# Autodesk Inventor assembly: final_Toolhead
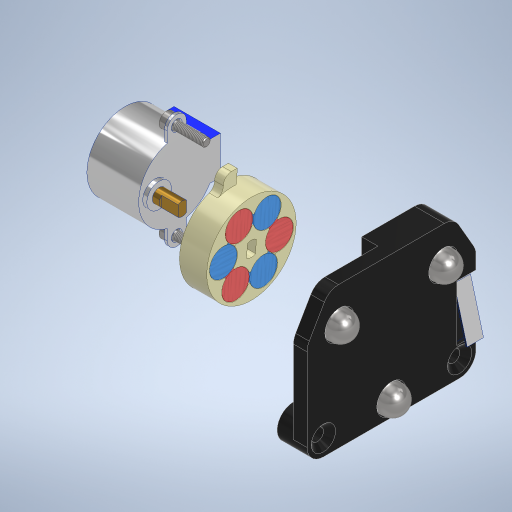
[picture p0: Inventor's stored thumbnail of the model, 512x512]
Saved by Autodesk Inventor 2023.2 (Build 272271000, 271)
## iProperties
Created: 2022-09-02
Part Number: final_Toolhead
Document SubType Name: Assembly
Designer: Remo
Author: Remo
## Documents named in this file (11)
- C:\Users\remop\OneDrive\Documents\Inventor\3D Printers\LuEVO\Mk4_Toolchanger\final_Toolhead.iam
- C:\Users\remop\OneDrive\Documents\Inventor\3D Printers\LuEVO\Mk4_Toolchanger\MagToolChanger_Lockplate.ipt
- C:\Users\remop\OneDrive\Documents\Inventor\3D Printers\LuEVO\Mk4_Toolchanger\MagToolChanger_HeadBase.ipt
- C:\Users\remop\OneDrive\Documents\Inventor\3D Printers\LuEVO\Mk4_Toolchanger\MagToolChanger_Motor.ipt
- C:\Users\remop\OneDrive\Documents\Inventor\3D Printers\LuEVO\Mk4_Toolchanger\MagToolChanger_RefSwitch.ipt
- C:\Users\remop\OneDrive\Documents\Inventor\3D Printers\LuEVO\Mk4_Toolchanger\MagToolChanger_Magnet.ipt
- C:\Users\remop\OneDrive\Documents\Inventor\3D Printers\LuEVO\Mk4_Toolchanger\MagToolChanger_CouplerBall.ipt
- C:\Users\remop\OneDrive\Documents\Inventor\Content Center Files\R2023\en-US\AS 1420\AS 1420 - 1973 - M3 x 12.ipt
- C:\Users\remop\OneDrive\Documents\Inventor\Content Center Files\R2023\en-US\ANSI B18.3.1M(6)\ANSI B18.3.1M - M2x0.4 x 10(1).ipt
- C:\Users\remop\OneDrive\Documents\Inventor\Content Center Files\R2023\en-US\AS 1420\AS 1420 - 1973 - M4 x 8.ipt
- C:\Users\remop\OneDrive\Documents\Inventor\Content Center Files\R2023\en-US\ANSI B18.3.4M(1)\ANSI B18.3.4M - M4 x 0.7 x 8(2).ipt
## Components (20 placed, 10 different names)
1. MagToolChanger_Lockplate:1 — Rigid:1, Rigid:2, Rigid:3, Rigid:4, Rigid:5, Rigid:6, Rotational:1
2. MagToolChanger_HeadBase:1 — Rigid:7, Rigid:8, Rigid:9, Rigid:10, Rigid:11, Insert:5, Insert:7, Insert:8
3. MagToolChanger_Motor:1 — Rotational:1, Rigid:11, Insert:1, Insert:2
4. MagToolChanger_RefSwitch:1 — Rigid:7, Insert:3, Insert:4
5. MagToolChanger_Magnet:1 — Rigid:6
6. MagToolChanger_Magnet:2 — Rigid:5
7. MagToolChanger_Magnet:3 — Rigid:3
8. MagToolChanger_Magnet:4 — Rigid:4
9. MagToolChanger_Magnet:5 — Rigid:2
10. MagToolChanger_Magnet:6 — Rigid:1
11. MagToolChanger_CouplerBall:1 — Rigid:9
12. MagToolChanger_CouplerBall:2 — Rigid:10
13. MagToolChanger_CouplerBall:3 — Rigid:8
14. AS 1420 - Metric M3 x 12:1 — Insert:1
15. AS 1420 - Metric M3 x 12:2 — Insert:2
16. Forged Socket Head Cap Screw - Metric M2x0.4 x 10:1 — Insert:3
17. Forged Socket Head Cap Screw - Metric M2x0.4 x 10:2 — Insert:4
18. AS 1420 - Metric M4 x 8:1 — Insert:5
19. AS 1420 - Metric M4 x 8:3 — Insert:7
20. Broached Hexagon Socket Button Head Cap Screw - Metric M4 x 0.7 x 8:1 — Insert:8
## Relationships (19: WeldJoint 11, Insert 7, RevoluteJoint 1)
- Rigid:1 [WeldJoint]: MagToolChanger_Lockplate:1 ↔ MagToolChanger_Magnet:6
- Rigid:2 [WeldJoint]: MagToolChanger_Lockplate:1 ↔ MagToolChanger_Magnet:5
- Rigid:3 [WeldJoint]: MagToolChanger_Lockplate:1 ↔ MagToolChanger_Magnet:3
- Rigid:4 [WeldJoint]: MagToolChanger_Lockplate:1 ↔ MagToolChanger_Magnet:4
- Rigid:5 [WeldJoint]: MagToolChanger_Lockplate:1 ↔ MagToolChanger_Magnet:2
- Rigid:6 [WeldJoint]: MagToolChanger_Lockplate:1 ↔ MagToolChanger_Magnet:1
- Rigid:7 [WeldJoint]: MagToolChanger_HeadBase:1 ↔ MagToolChanger_RefSwitch:1
- Rigid:8 [WeldJoint]: MagToolChanger_HeadBase:1 ↔ MagToolChanger_CouplerBall:3
- Rigid:9 [WeldJoint]: MagToolChanger_HeadBase:1 ↔ MagToolChanger_CouplerBall:1
- Rigid:10 [WeldJoint]: MagToolChanger_HeadBase:1 ↔ MagToolChanger_CouplerBall:2
- Rotational:1 [RevoluteJoint] (-25.4 mm): MagToolChanger_Lockplate:1 ↔ MagToolChanger_Motor:1
- Rigid:11 [WeldJoint] (76.2 mm): MagToolChanger_HeadBase:1 ↔ MagToolChanger_Motor:1
- Insert:1: MagToolChanger_Motor:1 ↔ AS 1420 - Metric M3 x 12:1
- Insert:2: MagToolChanger_Motor:1 ↔ AS 1420 - Metric M3 x 12:2
- Insert:3: MagToolChanger_RefSwitch:1 ↔ Forged Socket Head Cap Screw - Metric M2x0.4 x 10:1
- Insert:4: MagToolChanger_RefSwitch:1 ↔ Forged Socket Head Cap Screw - Metric M2x0.4 x 10:2
- Insert:5: MagToolChanger_HeadBase:1 ↔ AS 1420 - Metric M4 x 8:1
- Insert:7: MagToolChanger_HeadBase:1 ↔ AS 1420 - Metric M4 x 8:3
- Insert:8: MagToolChanger_HeadBase:1 ↔ Broached Hexagon Socket Button Head Cap Screw - Metric M4 x 0.7 x 8:1
